# Autodesk Inventor assembly: 110-01
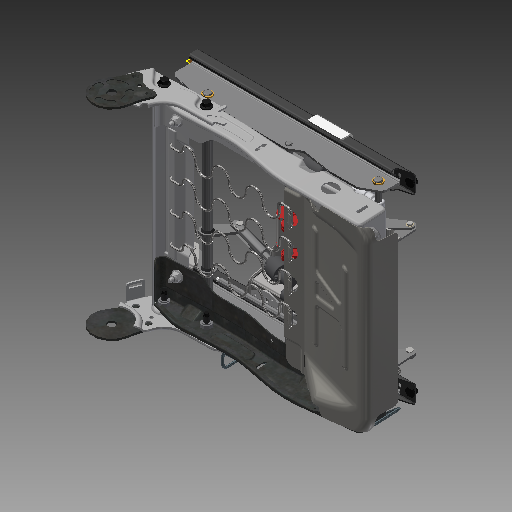
[picture p0: Inventor's stored thumbnail of the model, 512x512]
Saved by Autodesk Inventor 2019 (Build 230136000, 136)
## iProperties
Company: Autodesk Inc.
Created: 2007-12-24
Part Number: 110-01
Document SubType Name: Assembly
Designer: Autodesk Inc.
Mass: 12502.3 g
Surface Area: 15972.1 cm^2
Volume: 1865.58 cm^3
Density: 6.70157 g/cm^3
Description: LOWER FULL ASSEMBLY
Component Category: Lower Component
Author: Inventor
## Documents named in this file (21)
- C:\TEMP\Car Seat\Workspace\Lower Full Assembly.iam
- C:\TEMP\Car Seat\Workspace\Bottom Guide Rail Assembly.iam
- C:\TEMP\Car Seat\Workspace\Front Pivot Links.iam
- C:\TEMP\Car Seat\Workspace\Pivot Plate.ipt
- C:\TEMP\Car Seat\Workspace\Pivot Link Weldment.iam
- C:\TEMP\Car Seat\Workspace\Top Frame Assembly.iam
- C:\TEMP\Car Seat\Workspace\Ball Screw Sleeve.ipt
- C:\TEMP\Car Seat\Workspace\Pivot Pin A.ipt
- C:\TEMP\Car Seat\Workspace\Worm Gear Housing.ipt
- C:\TEMP\Car Seat\Workspace\Ball Screw Shaft B.ipt
- C:\TEMP\Car Seat\Workspace\Motor.iam
- C:\TEMP\Car Seat\Workspace\Pivot Rod.ipt
- C:\TEMP\Car Seat\Workspace\Back Support Plate R.ipt
- C:\TEMP\Car Seat\Workspace\Back Support Plate L.ipt
- C:\TEMP\Car Seat\Workspace\Side Pivot Plate.ipt
- C:\TEMP\Car Seat\Workspace\Top Platform Mounting Bolt.ipt
- C:\TEMP\Car Seat\Workspace\Top Platform Mounting Nut.ipt
- C:\TEMP\Car Seat\Workspace\Front Worm Drive Assembly.iam
- C:\TEMP\Car Seat\Workspace\Rear Worm Drive Assembly.iam
- C:\TEMP\Car Seat\Workspace\Bottom Rail Assembly.iam
- C:\TEMP\Car Seat\Workspace\Front Link.ipt
## Components (31 placed, 20 different names)
1. Bottom Rail Assembly:1 [sub-assembly] — Flush:7, Flush:8, Flush:9, Mate:2, Mate:5
2. Bottom Guide Rail Assembly:1 [sub-assembly] — Flush:10, Flush:11, Flush:12, Insert:2, Insert:4, Mate:3, Mate:11, Mate:34
3. Front Pivot Links:1 [sub-assembly] — Insert:2, Mate:1, Mate:6, Mate:10, Mate:15, Angle:1, Mate:31, Mate:32
4. Pivot Plate:1 — Mate:15, Mate:17, Mate:18, Angle:1
5. Pivot Link Weldment:1 [sub-assembly] — Insert:4, Mate:13, Mate:14, Mate:33
6. Top Frame Assembly:1 [sub-assembly] — Mate:33, Insert:8, Mate:25, Insert:12, Insert:13, Mate:26, Insert:17, Insert:19, Insert:20, Insert:21, Insert:22
7. Ball Screw Sleeve:1 — Mate:16, Mate:17, Mate:18, Mate:21, Tangent:1
8. Ball Screw Sleeve:2 — Mate:12, Mate:13, Mate:14
9. Pivot Pin A:1 — Mate:21, Tangent:1
10. Worm Gear Housing:1 — Mate:1, Mate:2, Insert:3
11. Worm Gear Housing:2 — Mate:5, Mate:6, Mate:7, Insert:18
12. Ball Screw Shaft B:1 — Insert:3
13. Ball Screw Shaft B:2 — Insert:18
14. Motor:1 [sub-assembly] — Mate:9, Mate:10
15. Pivot Rod:1 — Mate:7, Mate:8, Mate:9
16. Back Support Plate L:1 — Mate:22, Mate:23, Mate:24, Insert:8, Mate:25, Insert:9, Insert:10
17. Top Platform Mounting Bolt:2 — Insert:9
18. Top Platform Mounting Bolt:1 — Insert:10
19. Top Platform Mounting Nut:3 — Insert:21
20. Back Support Plate R:1 — Insert:13, Mate:26, Mate:27, Mate:28, Mate:29, Insert:14, Insert:15
21. Top Platform Mounting Nut:4 — Insert:12
22. Top Platform Mounting Bolt:3 — Insert:15
23. Top Platform Mounting Bolt:4 — Insert:14
24. Top Platform Mounting Nut:1 — Insert:22
25. Top Platform Mounting Nut:2 — Insert:17
26. Side Pivot Plate:2 — Mate:27, Mate:28, Mate:29
27. Side Pivot Plate:1 — Mate:22, Mate:23, Mate:24
28. Front Worm Drive Assembly:1 [sub-assembly] — Mate:3, Mate:16, Mate:30, Mate:11
29. Rear Worm Drive Assembly:1 [sub-assembly] — Mate:12, Mate:30, Mate:34
30. Front Link:1 — Mate:31, Insert:19
31. Front Link:2 — Mate:32, Insert:20
## Relationships (55: Mate 31, Insert 16, Flush 6, Tangent 1, Angle 1)
- Flush:7: Bottom Rail Assembly:1
- Flush:8: Bottom Rail Assembly:1
- Flush:9: Bottom Rail Assembly:1
- Flush:10: Bottom Guide Rail Assembly:1
- Flush:11: Bottom Guide Rail Assembly:1
- Flush:12: Bottom Guide Rail Assembly:1
- Insert:2: Bottom Guide Rail Assembly:1 ↔ Front Pivot Links:1
- Mate:1: Front Pivot Links:1 ↔ Worm Gear Housing:1
- Mate:2: Bottom Rail Assembly:1 ↔ Worm Gear Housing:1
- Insert:3: Worm Gear Housing:1 ↔ Ball Screw Shaft B:1
- Insert:4: Bottom Guide Rail Assembly:1 ↔ Pivot Link Weldment:1
- Mate:3: Bottom Guide Rail Assembly:1 ↔ Front Worm Drive Assembly:1
- Mate:5: Bottom Rail Assembly:1 ↔ Worm Gear Housing:2
- Mate:6: Front Pivot Links:1 ↔ Worm Gear Housing:2
- Mate:7: Worm Gear Housing:2 ↔ Pivot Rod:1
- Mate:8: Pivot Rod:1
- Mate:9: Motor:1 ↔ Pivot Rod:1
- Mate:10: Front Pivot Links:1 ↔ Motor:1
- Mate:11: Bottom Guide Rail Assembly:1 ↔ Front Worm Drive Assembly:1
- Mate:12: Ball Screw Sleeve:2 ↔ Rear Worm Drive Assembly:1
- Mate:13: Pivot Link Weldment:1 ↔ Ball Screw Sleeve:2
- Mate:14: Pivot Link Weldment:1 ↔ Ball Screw Sleeve:2
- Mate:15: Front Pivot Links:1 ↔ Pivot Plate:1
- Mate:16: Ball Screw Sleeve:1 ↔ Front Worm Drive Assembly:1
- Mate:17: Pivot Plate:1 ↔ Ball Screw Sleeve:1
- Mate:18: Pivot Plate:1 ↔ Ball Screw Sleeve:1
- Mate:33: Pivot Link Weldment:1 ↔ Top Frame Assembly:1
- Mate:21: Ball Screw Sleeve:1 ↔ Pivot Pin A:1
- Tangent:1: Ball Screw Sleeve:1 ↔ Pivot Pin A:1
- Angle:1 (100 deg): Front Pivot Links:1 ↔ Pivot Plate:1
- Mate:22: Back Support Plate L:1 ↔ Side Pivot Plate:1
- Mate:23: Back Support Plate L:1 ↔ Side Pivot Plate:1
- Mate:24: Back Support Plate L:1 ↔ Side Pivot Plate:1
- Insert:8: Top Frame Assembly:1 ↔ Back Support Plate L:1
- Mate:25: Top Frame Assembly:1 ↔ Back Support Plate L:1
- Insert:9: Back Support Plate L:1 ↔ Top Platform Mounting Bolt:2
- Insert:10: Back Support Plate L:1 ↔ Top Platform Mounting Bolt:1
- Insert:12: Top Frame Assembly:1 ↔ Top Platform Mounting Nut:4
- Insert:13: Top Frame Assembly:1 ↔ Back Support Plate R:1
- Mate:26: Top Frame Assembly:1 ↔ Back Support Plate R:1
- Mate:27: Back Support Plate R:1 ↔ Side Pivot Plate:2
- Mate:28: Back Support Plate R:1 ↔ Side Pivot Plate:2
- Mate:29: Back Support Plate R:1 ↔ Side Pivot Plate:2
- Insert:14: Back Support Plate R:1 ↔ Top Platform Mounting Bolt:4
- Insert:15: Back Support Plate R:1 ↔ Top Platform Mounting Bolt:3
- Insert:17: Top Frame Assembly:1 ↔ Top Platform Mounting Nut:2
- Mate:30: Front Worm Drive Assembly:1 ↔ Rear Worm Drive Assembly:1
- Insert:18: Worm Gear Housing:2 ↔ Ball Screw Shaft B:2
- Mate:31: Front Pivot Links:1 ↔ Front Link:1
- Insert:19: Top Frame Assembly:1 ↔ Front Link:1
- Mate:32: Front Pivot Links:1 ↔ Front Link:2
- Insert:20: Top Frame Assembly:1 ↔ Front Link:2
- Insert:21: Top Frame Assembly:1 ↔ Top Platform Mounting Nut:3
- Insert:22: Top Frame Assembly:1 ↔ Top Platform Mounting Nut:1
- Mate:34: Bottom Guide Rail Assembly:1 ↔ Rear Worm Drive Assembly:1
